# Autodesk Inventor assembly: internal-mount
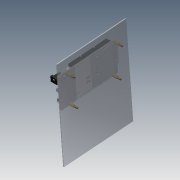
[picture p0: Inventor's stored thumbnail of the model, 180x180]
Saved by Autodesk Inventor 2015 SP1 (Build 190203100, 203)
## iProperties
Created: 2015-07-22
Part Number: internal-mount
Document SubType Name: Assembly
Designer: James
Author: James
## Documents named in this file (4)
- D:\James\Documents\Inventor\DFB Electronics box mount\internal-mount.iam
- D:\James\Documents\Inventor\DFB Electronics box mount\mount.ipt
- D:\James\Documents\Inventor\DFB Electronics box mount\arduino\Imported Components\ARDUINO DUE\ARDUINO DUE_JK.iam
- D:\James\Documents\Inventor\DFB Electronics box mount\standoff.ipt
## Components (6 placed, 3 different names)
1. mount:1 — Mate:1, Mate:2, Angle:1, Mate:3, Mate:4, Mate:5, Mate:6, Mate:7, Mate:8, Mate:9
2. ARDUINO DUE_JK:1 [sub-assembly] — Mate:2, Angle:1, Mate:10
3. standoff:1 — Mate:6, Mate:9
4. standoff:2 — Mate:5, Mate:7, Mate:10
5. standoff:3 — Mate:4, Mate:8
6. standoff:4 — Mate:1, Mate:3
## Relationships (11: Mate 10, Angle 1)
- Mate:1: mount:1 ↔ standoff:4
- Mate:2: mount:1 ↔ ARDUINO DUE_JK:1
- Angle:1 (180 deg): mount:1 ↔ ARDUINO DUE_JK:1
- Mate:3: mount:1 ↔ standoff:4
- Mate:4: mount:1 ↔ standoff:3
- Mate:5: mount:1 ↔ standoff:2
- Mate:6: mount:1 ↔ standoff:1
- Mate:7: mount:1 ↔ standoff:2
- Mate:8: mount:1 ↔ standoff:3
- Mate:9: mount:1 ↔ standoff:1
- Mate:10: ARDUINO DUE_JK:1 ↔ standoff:2
